# Autodesk Inventor assembly: Assembly1
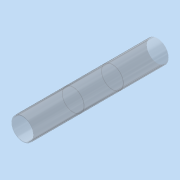
[picture p0: Inventor's stored thumbnail of the model, 180x180]
Saved by Autodesk Inventor 2017 (Build 210142000, 142)
## iProperties
Created: 2016-11-14
Part Number: Assembly1
Document SubType Name: Assembly
Designer: techn
Author: techn
## Documents named in this file (4)
- D:\OneDrive\Documents\Other Projects\Submarine\CAD\midships\test\pressureHullTest\Assembly1.iam
- D:\OneDrive\Documents\Other Projects\Submarine\CAD\midships\test\pressureHullTest\aftSection.ipt
- D:\OneDrive\Documents\Other Projects\Submarine\CAD\midships\test\pressureHullTest\foreSection.ipt
- D:\OneDrive\Documents\Other Projects\Submarine\CAD\midships\test\pressureHullTest\pressure section.ipt
## Components (3 placed, 3 different names)
1. aftSection:1 — Mate:2, Mate:4
2. foreSection:1 — Mate:1, Mate:3
3. pressure section:1 — Mate:1, Mate:2, Mate:3, Mate:4
## Relationships (4: Mate 4)
- Mate:1: foreSection:1 ↔ pressure section:1
- Mate:2: aftSection:1 ↔ pressure section:1
- Mate:3: foreSection:1 ↔ pressure section:1
- Mate:4: aftSection:1 ↔ pressure section:1
